# Autodesk Inventor assembly: montagem
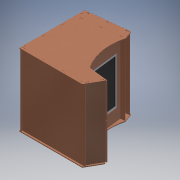
[picture p0: Inventor's stored thumbnail of the model, 180x180]
Saved by Autodesk Inventor 2017 (Build 210142000, 142)
## iProperties
Created: 2017-10-05
Part Number: montagem
Document SubType Name: Assembly
Designer: Felipe
Author: Felipe
## Documents named in this file (11)
- D:\Dropbox\Fliperama\montagem.iam
- D:\Dropbox\Fliperama\ladoA.ipt
- D:\Dropbox\Fliperama\Fundo.ipt
- D:\Dropbox\Fliperama\Base.ipt
- D:\Dropbox\Fliperama\Superior_top.ipt
- D:\Dropbox\Fliperama\Superior_3mm.ipt
- D:\Dropbox\Fliperama\Frente_Controle.ipt
- D:\Dropbox\Fliperama\TV.ipt
- D:\Dropbox\Fliperama\Frontal.ipt
- D:\Dropbox\Fliperama\joystick.ipt
- D:\Dropbox\Fliperama\bt.ipt
## Components (12 placed, 10 different names)
1. ladoA:1 — Mate:1, Flush:1, Mate:4, Mate:14, Mate:15, Mate:16, Mate:18, Mate:20, Flush:4
2. ladoA:2 — Mate:2, Flush:1, Mate:3, Mate:5, Mate:6, Mate:10, Mate:11, Mate:12, Mate:13, Mate:17, Mate:19, Mate:33
3. Fundo:1 — Mate:3, Mate:4, Mate:5, Mate:6, Mate:7, Mate:8, Mate:9, Mate:23
4. Base:1 — Mate:7, Mate:8, Mate:9
5. Superior_top:1 — Mate:10, Mate:11, Mate:12
6. Superior_3mm:1 — Mate:13, Mate:14, Mate:15, Mate:21
7. Frente_Controle:1 — Mate:16, Mate:17, Mate:18, Mate:25, Mate:31
8. TV:1 — Mate:19, Flush:2, Flush:7
9. Frontal:1 — Mate:20, Mate:21, Flush:2, Flush:7
10. joystick:1 — Mate:25, Mate:26, Mate:27, Mate:28, Mate:29, Mate:30, Mate:31, Mate:32, Mate:33
11. bt:1 — Mate:27, Mate:30, Mate:32
12. bt:2 — Mate:26, Mate:28, Mate:29
## Relationships (35: Mate 31, Flush 4)
- Mate:1: ladoA:1
- Mate:2: ladoA:2
- Flush:1: ladoA:1 ↔ ladoA:2
- Mate:3: ladoA:2 ↔ Fundo:1
- Mate:4: ladoA:1 ↔ Fundo:1
- Mate:5: ladoA:2 ↔ Fundo:1
- Mate:6: ladoA:2 ↔ Fundo:1
- Mate:7: Fundo:1 ↔ Base:1
- Mate:8: Fundo:1 ↔ Base:1
- Mate:9: Fundo:1 ↔ Base:1
- Mate:10: ladoA:2 ↔ Superior_top:1
- Mate:11: ladoA:2 ↔ Superior_top:1
- Mate:12: ladoA:2 ↔ Superior_top:1
- Mate:13: ladoA:2 ↔ Superior_3mm:1
- Mate:14: ladoA:1 ↔ Superior_3mm:1
- Mate:15: ladoA:1 ↔ Superior_3mm:1
- Mate:16: ladoA:1 ↔ Frente_Controle:1
- Mate:17: ladoA:2 ↔ Frente_Controle:1
- Mate:18: ladoA:1 ↔ Frente_Controle:1
- Mate:19 (50 mm): ladoA:2 ↔ TV:1
- Mate:20: ladoA:1 ↔ Frontal:1
- Mate:21: Superior_3mm:1 ↔ Frontal:1
- Flush:2 (3 mm): TV:1 ↔ Frontal:1
- Flush:4: ladoA:1
- Mate:23: Fundo:1
- Mate:25: Frente_Controle:1 ↔ joystick:1
- Flush:7 (22 mm): TV:1 ↔ Frontal:1
- Mate:26: joystick:1 ↔ bt:2
- Mate:27: joystick:1 ↔ bt:1
- Mate:28: joystick:1 ↔ bt:2
- Mate:29: joystick:1 ↔ bt:2
- Mate:30: joystick:1 ↔ bt:1
- Mate:31: Frente_Controle:1 ↔ joystick:1
- Mate:32: joystick:1 ↔ bt:1
- Mate:33: ladoA:2 ↔ joystick:1
